# Autodesk Inventor assembly: Electrical Feedthrough Collar
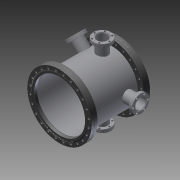
[picture p0: Inventor's stored thumbnail of the model, 180x180]
Saved by Autodesk Inventor 2014 (Build 180170000, 170)
## iProperties
Created: 2014-05-19
Part Number: Electrical Feedthrough Collar
Document SubType Name: Assembly
Designer: ijs09
Author: ijs09
## Documents named in this file (5)
- D:\Inventor\CCM CAD Files\CADFiles\Electrical Feedthrough Collar\Electrical Feedthrough Collar.iam
- D:\Inventor\CCM CAD Files\CADFiles\Electrical Feedthrough Collar\Vacuum Cylinder.ipt
- D:\Inventor\CCM CAD Files\CADFiles\Electrical Feedthrough Collar\DN200CF.ipt
- D:\Inventor\CCM CAD Files\CADFiles\Electrical Feedthrough Collar\DN35CF Counter Bored.ipt
- D:\Inventor\CCM CAD Files\CADFiles\Electrical Feedthrough Collar\DN16CF Counter Bored.ipt
## Components (9 placed, 4 different names)
1. Vacuum Cylinder:1 — Mate:1, Mate:2, Mate:3, Mate:4, Mate:5, Mate:6, Mate:7, Mate:8, Mate:9, Mate:10, Mate:11, Mate:12, Mate:13, Mate:14, Mate:15, Mate:16
2. DN200CF:1 — Mate:3, Mate:4
3. DN200CF:2 — Mate:1, Mate:2
4. DN35CF Counter Bored:1 — Mate:9, Mate:10
5. DN35CF Counter Bored:2 — Mate:7, Mate:8
6. DN35CF Counter Bored:3 — Mate:5, Mate:6
7. DN16CF Counter Bored:1 — Mate:11, Mate:12
8. DN35CF Counter Bored:4 — Mate:15, Mate:16
9. DN35CF Counter Bored:5 — Mate:13, Mate:14
## Relationships (16: Mate 16)
- Mate:1: Vacuum Cylinder:1 ↔ DN200CF:2
- Mate:2: Vacuum Cylinder:1 ↔ DN200CF:2
- Mate:3: Vacuum Cylinder:1 ↔ DN200CF:1
- Mate:4: Vacuum Cylinder:1 ↔ DN200CF:1
- Mate:5: Vacuum Cylinder:1 ↔ DN35CF Counter Bored:3
- Mate:6: Vacuum Cylinder:1 ↔ DN35CF Counter Bored:3
- Mate:7: Vacuum Cylinder:1 ↔ DN35CF Counter Bored:2
- Mate:8: Vacuum Cylinder:1 ↔ DN35CF Counter Bored:2
- Mate:9: Vacuum Cylinder:1 ↔ DN35CF Counter Bored:1
- Mate:10: Vacuum Cylinder:1 ↔ DN35CF Counter Bored:1
- Mate:11: Vacuum Cylinder:1 ↔ DN16CF Counter Bored:1
- Mate:12: Vacuum Cylinder:1 ↔ DN16CF Counter Bored:1
- Mate:13: Vacuum Cylinder:1 ↔ DN35CF Counter Bored:5
- Mate:14: Vacuum Cylinder:1 ↔ DN35CF Counter Bored:5
- Mate:15: Vacuum Cylinder:1 ↔ DN35CF Counter Bored:4
- Mate:16: Vacuum Cylinder:1 ↔ DN35CF Counter Bored:4
